# Autodesk Inventor assembly: Robot!
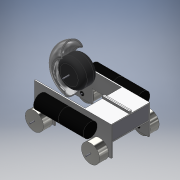
[picture p0: Inventor's stored thumbnail of the model, 180x180]
Saved by Autodesk Inventor 2016 (Build 200138000, 138)
## iProperties
Created: 2015-11-03
Part Number: Robot!
Document SubType Name: Assembly
Designer: rossmosier
Author: rossmosier
## Documents named in this file (5)
- C:\Users\rossmosier\Documents\CAD Team\CADTeam\Assemblies\Robot!.iam
- C:\Users\rossmosier\Documents\CAD Team\CADTeam\Parts\Brain.ipt
- C:\Users\rossmosier\Documents\CAD Team\CADTeam\Drive Train\driveAssembly.iam
- C:\Users\rossmosier\Documents\CAD Team\CADTeam\Drive Train\driveAssembly_MIR.iam
- C:\Users\rossmosier\Documents\CAD Team\CADTeam\Thrower\throwerAssembly.iam
## Components (4 placed, 4 different names)
1. Brain:1 — Mate:1, Mate:2
2. driveAssembly:1 [sub-assembly] — Mate:1
3. driveAssembly_MIR:1 [sub-assembly] — Mate:2
4. throwerAssembly:1 [sub-assembly]
## Relationships (2: Mate 2)
- Mate:1: Brain:1 ↔ driveAssembly:1
- Mate:2: Brain:1 ↔ driveAssembly_MIR:1
